# Autodesk Inventor assembly: elbowassembly
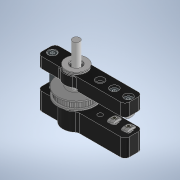
[picture p0: Inventor's stored thumbnail of the model, 180x180]
Saved by Autodesk Inventor 2022 (Build 260153000, 153)
## iProperties
Created: 2022-02-22
Part Number: elbowassembly
Document SubType Name: Assembly
Designer: JK
Author: JK
## Documents named in this file (14)
- C:\Users\JK\Documents\Inventor\ScaraNema\SCARA-3DP\Parts\Arm\Elbow assembly.iam
- C:\Users\JK\Documents\Inventor\ScaraNema\SCARA-3DP\Parts\Common components\GT260T.ipt
- C:\Users\JK\Documents\Inventor\ScaraNema\SCARA-3DP\Parts\Arm\Top pulley support.ipt
- C:\Users\JK\Documents\Inventor\ScaraNema\SCARA-3DP\Parts\Arm\Bottom pulley support.ipt
- C:\Users\JK\Documents\Inventor\ScaraNema\SCARA-3DP\Parts\Arm\8x80 mm axis.ipt
- C:\Users\JK\Documents\Inventor\ScaraNema\SCARA-3DP\Parts\Fasteners\M5 Hex nut.ipt
- C:\Users\JK\Documents\Inventor\ScaraNema\SCARA-3DP\Parts\Fasteners\M5x15 Flat head bolt.ipt
- C:\Users\JK\Documents\Inventor\ScaraNema\SCARA-3DP\Parts\Fasteners\M5 T-Nut Drop-in 20x20.ipt
- C:\Users\JK\Documents\Inventor\ScaraNema\SCARA-3DP\Parts\Fasteners\M5x25 Flat head bolt.ipt
- C:\Users\JK\Documents\Inventor\ScaraNema\SCARA-3DP\Parts\Fasteners\M5x55 Flat head bolt.ipt
- C:\Users\JK\Documents\Inventor\ScaraNema\SCARA-3DP\Parts\Arm\7806K712_Thrust Ball Bearing.ipt
- C:\Users\JK\Documents\Inventor\ScaraNema\SCARA-3DP\Parts\Arm\5909K31_Needle-Roller Thrust Bearing.ipt
- C:\Users\JK\Documents\Inventor\ScaraNema\SCARA-3DP\Parts\Arm\5909K44_0.032 Thick Washer for 1 2 Shaft Diameter Needle-Roller Thrust Bearing.ipt
- C:\Users\JK\Documents\Inventor\ScaraNema\SCARA-3DP\Parts\Common components\688-2RS.ipt
## Components (20 placed, 13 different names)
1. GT260T:1 — Coincidencia:24
2. Bottom pulley support:1 — Coincidencia:24, Coincidencia:29, Coincidencia:31, Ángulo:1, Coincidencia:32, Nivelación:2, Coincidencia:40, Coincidencia:41, Coincidencia:42, Coincidencia:45, Nivelación:6, Coincidencia:48, Coincidencia:49, Coincidencia:57
3. Top pulley support:1 — Coincidencia:29, Coincidencia:33, Coincidencia:34, Coincidencia:35, Coincidencia:36, Nivelación:2, Ángulo:3, Coincidencia:39, Coincidencia:46, Coincidencia:51, Coincidencia:54, Coincidencia:55, Coincidencia:58
4. 8x80 mm axis:1 — Coincidencia:36, Nivelación:6, Coincidencia:50, Coincidencia:52, Coincidencia:53, Coincidencia:56
5. M5 Hex nut:2 — Coincidencia:31, Ángulo:1, Coincidencia:32
6. M5x15 Flat head bolt:1 — Coincidencia:34, Nivelación:1, Coincidencia:35, Coincidencia:37
7. M5x15 Flat head bolt:2 — Coincidencia:33, Nivelación:1, Coincidencia:38
8. M5 T-Nut Drop-in 20x20:1 — Coincidencia:38, Ángulo:2, Nivelación:3, Coincidencia:39, Ángulo:5
9. M5 T-Nut Drop-in 20x20:2 — Coincidencia:37, Ángulo:2, Ángulo:3, Nivelación:3
10. M5x25 Flat head bolt:1 — Coincidencia:41, Nivelación:4, Coincidencia:42, Coincidencia:43
11. M5x25 Flat head bolt:2 — Coincidencia:40, Nivelación:4, Coincidencia:44
12. M5 T-Nut Drop-in 20x20:3 — Coincidencia:44, Nivelación:5, Ángulo:4, Ángulo:5, Coincidencia:45
13. M5 T-Nut Drop-in 20x20:4 — Coincidencia:43, Nivelación:5, Ángulo:4
14. M5x55 Flat head bolt:1 — Coincidencia:46, Coincidencia:58
15. 7806K712_Thrust Ball Bearing:1 — Coincidencia:48, Coincidencia:49
16. 5909K31_Needle-Roller Thrust Bearing:1 — Coincidencia:52, Tangente:1, Tangente:2
17. 5909K44_0.032 Thick Washer for 1 2 Shaft Diameter Needle-Roller Thrust Bearing:1 — Coincidencia:50, Coincidencia:51, Tangente:1
18. 5909K44_0.032 Thick Washer for 1 2 Shaft Diameter Needle-Roller Thrust Bearing:2 — Tangente:2, Coincidencia:53
19. 688-2RS:1 — Coincidencia:54, Coincidencia:55
20. 688-2RS:2 — Coincidencia:56, Coincidencia:57
## Relationships (42: Mate 29, Flush 6, Angle 5, Tangent 2)
- Coincidencia:24 [Mate] (7 mm): GT260T:1 ↔ Bottom pulley support:1
- Coincidencia:29 [Mate]: Bottom pulley support:1 ↔ Top pulley support:1
- Coincidencia:31 [Mate]: Bottom pulley support:1 ↔ M5 Hex nut:2
- Ángulo:1 [Angle] (0 deg): Bottom pulley support:1 ↔ M5 Hex nut:2
- Coincidencia:32 [Mate]: Bottom pulley support:1 ↔ M5 Hex nut:2
- Coincidencia:33 [Mate]: Top pulley support:1 ↔ M5x15 Flat head bolt:2
- Coincidencia:34 [Mate]: Top pulley support:1 ↔ M5x15 Flat head bolt:1
- Nivelación:1 [Flush]: M5x15 Flat head bolt:1 ↔ M5x15 Flat head bolt:2
- Coincidencia:35 [Mate]: Top pulley support:1 ↔ M5x15 Flat head bolt:1
- Coincidencia:36 [Mate]: Top pulley support:1 ↔ 8x80 mm axis:1
- Nivelación:2 [Flush]: Bottom pulley support:1 ↔ Top pulley support:1
- Coincidencia:37 [Mate]: M5x15 Flat head bolt:1 ↔ M5 T-Nut Drop-in 20x20:2
- Coincidencia:38 [Mate]: M5x15 Flat head bolt:2 ↔ M5 T-Nut Drop-in 20x20:1
- Ángulo:2 [Angle] (0 deg): M5 T-Nut Drop-in 20x20:1 ↔ M5 T-Nut Drop-in 20x20:2
- Ángulo:3 [Angle] (90 deg): Top pulley support:1 ↔ M5 T-Nut Drop-in 20x20:2
- Nivelación:3 [Flush]: M5 T-Nut Drop-in 20x20:1 ↔ M5 T-Nut Drop-in 20x20:2
- Coincidencia:39 [Mate] (0.6 mm): Top pulley support:1 ↔ M5 T-Nut Drop-in 20x20:1
- Coincidencia:40 [Mate]: Bottom pulley support:1 ↔ M5x25 Flat head bolt:2
- Coincidencia:41 [Mate]: Bottom pulley support:1 ↔ M5x25 Flat head bolt:1
- Nivelación:4 [Flush]: M5x25 Flat head bolt:1 ↔ M5x25 Flat head bolt:2
- Coincidencia:42 [Mate]: Bottom pulley support:1 ↔ M5x25 Flat head bolt:1
- Coincidencia:43 [Mate]: M5x25 Flat head bolt:1 ↔ M5 T-Nut Drop-in 20x20:4
- Coincidencia:44 [Mate]: M5x25 Flat head bolt:2 ↔ M5 T-Nut Drop-in 20x20:3
- Nivelación:5 [Flush]: M5 T-Nut Drop-in 20x20:3 ↔ M5 T-Nut Drop-in 20x20:4
- Ángulo:4 [Angle] (0 deg): M5 T-Nut Drop-in 20x20:3 ↔ M5 T-Nut Drop-in 20x20:4
- Ángulo:5 [Angle] (0 deg): M5 T-Nut Drop-in 20x20:1 ↔ M5 T-Nut Drop-in 20x20:3
- Coincidencia:45 [Mate] (0.6 mm): Bottom pulley support:1 ↔ M5 T-Nut Drop-in 20x20:3
- Nivelación:6 [Flush]: Bottom pulley support:1 ↔ 8x80 mm axis:1
- Coincidencia:46 [Mate]: Top pulley support:1 ↔ M5x55 Flat head bolt:1
- Coincidencia:48 [Mate]: Bottom pulley support:1 ↔ 7806K712_Thrust Ball Bearing:1
- Coincidencia:49 [Mate]: Bottom pulley support:1 ↔ 7806K712_Thrust Ball Bearing:1
- Coincidencia:50 [Mate]: 8x80 mm axis:1 ↔ 5909K44_0.032 Thick Washer for 1 2 Shaft Diameter Needle-Roller Thrust Bearing:1
- Coincidencia:51 [Mate]: Top pulley support:1 ↔ 5909K44_0.032 Thick Washer for 1 2 Shaft Diameter Needle-Roller Thrust Bearing:1
- Coincidencia:52 [Mate]: 8x80 mm axis:1 ↔ 5909K31_Needle-Roller Thrust Bearing:1
- Tangente:1: 5909K31_Needle-Roller Thrust Bearing:1 ↔ 5909K44_0.032 Thick Washer for 1 2 Shaft Diameter Needle-Roller Thrust Bearing:1
- Tangente:2: 5909K31_Needle-Roller Thrust Bearing:1 ↔ 5909K44_0.032 Thick Washer for 1 2 Shaft Diameter Needle-Roller Thrust Bearing:2
- Coincidencia:53 [Mate]: 8x80 mm axis:1 ↔ 5909K44_0.032 Thick Washer for 1 2 Shaft Diameter Needle-Roller Thrust Bearing:2
- Coincidencia:54 [Mate]: Top pulley support:1 ↔ 688-2RS:1
- Coincidencia:55 [Mate]: Top pulley support:1 ↔ 688-2RS:1
- Coincidencia:56 [Mate]: 8x80 mm axis:1 ↔ 688-2RS:2
- Coincidencia:57 [Mate]: Bottom pulley support:1 ↔ 688-2RS:2
- Coincidencia:58 [Mate]: Top pulley support:1 ↔ M5x55 Flat head bolt:1
